# Autodesk Inventor assembly: Montagem1
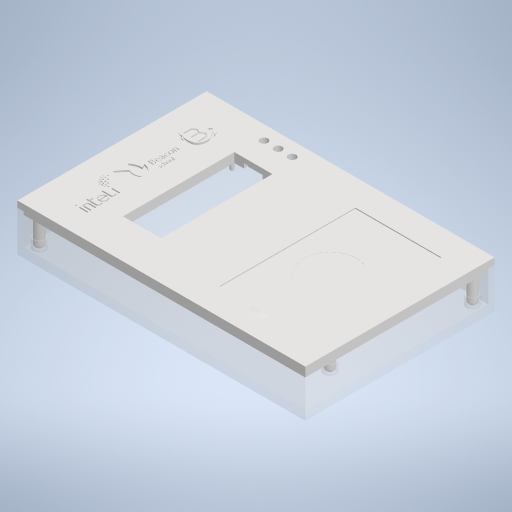
[picture p0: Inventor's stored thumbnail of the model, 512x512]
Saved by Autodesk Inventor 2023 (Build 270158000, 158)
## iProperties
Created: 2022-11-25
Part Number: Montagem1
Document SubType Name: Assembly
Designer: Inteli
Author: Inteli
## Documents named in this file (3)
- C:\Users\Inteli\Documents\GitHub\Projeto3\src\Inventor - Protótipo da CAse\Montagem\Montagem1.iam
- C:\Users\Inteli\Documents\GitHub\Projeto3\src\Inventor - Protótipo da CAse\Peças\base_traseira.ipt
- C:\Users\Inteli\Documents\GitHub\Projeto3\src\Inventor - Protótipo da CAse\Peças\Case Oficial.ipt
## Components (2 placed, 2 different names)
1. base_traseira:1 — Alinhado:1, Alinhado:2, Coincidente:1
2. Case Oficial:1 — Alinhado:1, Alinhado:2, Coincidente:1
## Relationships (3: Flush 2, Mate 1)
- Alinhado:1 [Flush]: base_traseira:1 ↔ Case Oficial:1
- Alinhado:2 [Flush]: base_traseira:1 ↔ Case Oficial:1
- Coincidente:1 [Mate]: base_traseira:1 ↔ Case Oficial:1
